# Autodesk Inventor assembly: flag edit
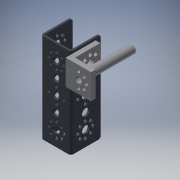
[picture p0: Inventor's stored thumbnail of the model, 180x180]
Saved by Autodesk Inventor 2016 (Build 200138000, 138)
## iProperties
Created: 2016-01-18
Part Number: flag edit
Document SubType Name: Assembly
Designer: tbloo
Author: tbloo
## Documents named in this file (3)
- C:\Users\tbloo\Documents\GitHub\phi_robotics\3d-models\FTC_Tetrix_KOP_Block_Party\Tim Bloot Designs\flag edit.iam
- C:\Users\tbloo\Documents\GitHub\phi_robotics\3d-models\FTC_Tetrix_KOP_Block_Party\Tim Bloot Designs\Flag Mount.ipt
- C:\Users\tbloo\Documents\GitHub\phi_robotics\3d-models\FTC_Tetrix_KOP_Block_Party\Tetrix_Kit_FTC\Autodesk Inventor Files\tetrix_c_channel-2.ipt
## Components (2 placed, 2 different names)
1. Flag Mount:1 — Rigid:1
2. tetrix_c_channel-2:1 — Rigid:1
## Relationships (1: WeldJoint 1)
- Rigid:1 [WeldJoint]: Flag Mount:1 ↔ tetrix_c_channel-2:1
